# Autodesk Inventor assembly: FrontBumper_Assembly
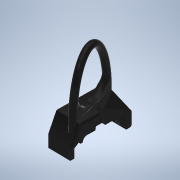
[picture p0: Inventor's stored thumbnail of the model, 180x180]
Saved by Autodesk Inventor 2020 (Build 240168000, 168)
## iProperties
Created: 2019-05-01
Part Number: FrontBumper_Assembly
Material: 一般
Document SubType Name: Assembly
Designer: taka
Mass: 15.5211 g
Surface Area: 61.7089 cm^2
Volume: 12.1259 cm^3
Density: 1.28 g/cm^3
Author: taka
## Documents named in this file (3)
- C:\Users\taka\Documents\GitHub\OpenPlatform\mechanism\OpenPlatform_ver3_0\上半身\胴体\FrontBumper.iam
- C:\Users\taka\Documents\GitHub\OpenPlatform\mechanism\OpenPlatform_ver3_0\上半身\胴体\FreundBumper_Stand.ipt
- C:\Users\taka\Documents\GitHub\OpenPlatform\mechanism\OpenPlatform_ver3_0\上半身\胴体\FrontBumper_main.ipt
## Components (2 placed, 2 different names)
1. FreundBumper_Stand:1 — メイト:2, 挿入:1
2. FrontBumper_main:1 — メイト:2, 挿入:1
## Relationships (2: Mate 1, Insert 1)
- メイト:2 [Mate] (0.1 mm): FreundBumper_Stand:1 ↔ FrontBumper_main:1
- 挿入:1 [Insert]: FreundBumper_Stand:1 ↔ FrontBumper_main:1
